# Autodesk Inventor assembly: XY Joint Left (Tulip)
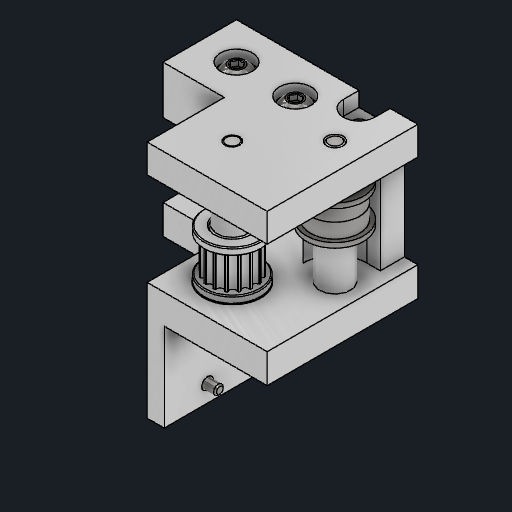
[picture p0: Inventor's stored thumbnail of the model, 512x512]
Saved by Autodesk Inventor 2026.1 (Build 301233020, 233B)
## iProperties
Created: 2025-05-24
Part Number: XY Joint Left (Tulip)
Document SubType Name: Assembly
Designer: Joshua Eah
Author: Joshua Eah
## Documents named in this file (9)
- C:\Users\JoshuaEah\Documents\GitHub\Voron-0\CAD\Tulip - Machined Parts\XY Joints\XY Joint Right\XY Joint Right (Tulip).iam
- C:\Users\JoshuaEah\Documents\GitHub\Voron-0\CAD\Tulip - Machined Parts\XY Joints\XY Joint Right\XY Joint Right Upper (Tulip).ipt
- C:\Users\JoshuaEah\Documents\GitHub\Voron-0\CAD\Tulip - Machined Parts\XY Joints\XY Joint Right\XY Joint Right Lower (Tulip).ipt
- C:\Users\JoshuaEah\Documents\GitHub\Voron-0\CAD\Master Assembly\Hardware\M3x6 BHCS.ipt
- C:\Users\JoshuaEah\Documents\GitHub\Voron-0\CAD\Master Assembly\Hardware\M3x12 BHCS.ipt
- C:\Users\JoshuaEah\Documents\GitHub\Voron-0\CAD\Master Assembly\Hardware\M2x6 FHCS.ipt
- C:\Users\JoshuaEah\Documents\GitHub\Voron-0\CAD\Tulip - Machined Parts\XY Joints\XY Joint Right\Right Idler Stack.iam
- C:\Users\JoshuaEah\Documents\GitHub\Voron-0\CAD\Tulip - Machined Parts\XY Joints\XY Joint Right\Right Pulley Stack.iam
- C:\Users\JoshuaEah\Documents\GitHub\Voron-0\CAD\Tulip - Machined Parts\XY Joints\Spacers\Joint Spacer.ipt
## Components (12 placed, 8 different names)
1. XY Joint Right Upper (Tulip):1 — Insert:20, Insert:21, Mate:1, Mate:4, Mate:5, Mate:6, Insert:34
2. XY Joint Right Lower (Tulip):1 — Insert:19, Insert:22, Insert:23, Insert:24, Insert:25, Insert:33
3. Right Idler Stack:1 [sub-assembly] — Mate:1
4. Right Pulley Stack:1 [sub-assembly] — Mate:5, Mate:6
5. M3x6 BHCS:1 — Insert:19
6. M3x12 BHCS:1 — Insert:20
7. M3x12 BHCS:2 — Insert:21
8. M2x6 FHCS:1 — Insert:22
9. M2x6 FHCS:2 — Insert:23
10. M2x6 FHCS:3 — Insert:24
11. M2x6 FHCS:4 — Insert:25
12. Joint Spacer:1 — Mate:4, Insert:33, Insert:34
## Relationships (18: Insert 10, Mate 6, Flush 2)
- Insert:19: XY Joint Right Lower (Tulip):1 ↔ M3x6 BHCS:1
- Insert:20: XY Joint Right Upper (Tulip):1 ↔ M3x12 BHCS:1
- Insert:21: XY Joint Right Upper (Tulip):1 ↔ M3x12 BHCS:2
- Insert:22: XY Joint Right Lower (Tulip):1 ↔ M2x6 FHCS:1
- Insert:23: XY Joint Right Lower (Tulip):1 ↔ M2x6 FHCS:2
- Insert:24: XY Joint Right Lower (Tulip):1 ↔ M2x6 FHCS:3
- Insert:25: XY Joint Right Lower (Tulip):1 ↔ M2x6 FHCS:4
- [Insert]: XY Joint Right Lower (Tulip):1 ↔ Right Idler Stack:1
- [Flush]: XY Joint Right Upper (Tulip):1 ↔ Right Idler Stack:1
- Mate:1: XY Joint Right Upper (Tulip):1 ↔ Right Idler Stack:1
- [Mate]: XY Joint Right Lower (Tulip):1 ↔ Right Pulley Stack:1
- [Mate]: XY Joint Right Lower (Tulip):1 ↔ Right Pulley Stack:1
- [Flush]: XY Joint Right Upper (Tulip):1 ↔ Right Pulley Stack:1
- Mate:4: XY Joint Right Upper (Tulip):1 ↔ Joint Spacer:1
- Mate:5: XY Joint Right Upper (Tulip):1 ↔ Right Pulley Stack:1
- Mate:6: XY Joint Right Upper (Tulip):1 ↔ Right Pulley Stack:1
- Insert:33: XY Joint Right Lower (Tulip):1 ↔ Joint Spacer:1
- Insert:34: XY Joint Right Upper (Tulip):1 ↔ Joint Spacer:1
